# Autodesk Inventor assembly: Shim_Assem_V5
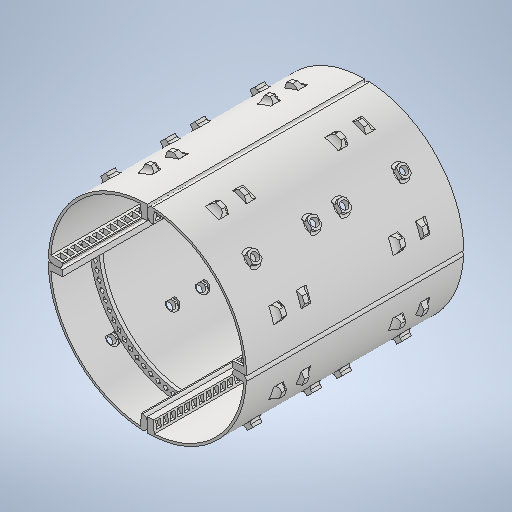
[picture p0: Inventor's stored thumbnail of the model, 512x512]
Saved by Autodesk Inventor 2025.2 (Build 292293000, 293)
## iProperties
Created: 2025-04-14
Part Number: Shim_Assem_V5
Document SubType Name: Assembly
Designer: Joshua Harper
Author: Joshua Harper
## Documents named in this file (3)
- C:\Users\Carla Fernandez\Documents\GitHub\OSII_MINI_V2\CAD MODELS\Shim_Assem_V5.iam
- C:\Users\Carla Fernandez\Documents\GitHub\OSII_MINI_V2\CAD MODELS\shim_tray_V5.ipt
- C:\Users\Carla Fernandez\Documents\GitHub\OSII_MINI_V2\CAD MODELS\shim_cartridge_V4.ipt
## Components (5 placed, 2 different names)
1. shim_tray_V5:1 — Mate:1, Flush:1, Tangent:1, Tangent:3, Flush:4, Flush:5, Flush:6
2. shim_tray_V5:2 — Mate:1, Flush:1, Tangent:1, Mate:2, Flush:2, Tangent:2, Mate:4, Mate:5
3. shim_tray_V5:3 — Mate:2, Flush:2, Tangent:2, Mate:3, Flush:3
4. shim_tray_V5:4 — Mate:3, Flush:3, Tangent:3
5. shim_cartridge_V4:1 — Mate:4, Mate:5
## Relationships (14: Flush 6, Mate 5, Tangent 3)
- Mate:1: shim_tray_V5:1 ↔ shim_tray_V5:2
- Flush:1: shim_tray_V5:1 ↔ shim_tray_V5:2
- Tangent:1: shim_tray_V5:1 ↔ shim_tray_V5:2
- Mate:2: shim_tray_V5:2 ↔ shim_tray_V5:3
- Flush:2: shim_tray_V5:2 ↔ shim_tray_V5:3
- Tangent:2: shim_tray_V5:2 ↔ shim_tray_V5:3
- Mate:3: shim_tray_V5:3 ↔ shim_tray_V5:4
- Flush:3: shim_tray_V5:3 ↔ shim_tray_V5:4
- Tangent:3: shim_tray_V5:1 ↔ shim_tray_V5:4
- Mate:4: shim_tray_V5:2 ↔ shim_cartridge_V4:1
- Mate:5: shim_tray_V5:2 ↔ shim_cartridge_V4:1
- Flush:4: shim_tray_V5:1
- Flush:5: shim_tray_V5:1
- Flush:6: shim_tray_V5:1
